# Autodesk Inventor assembly: SE Base Matriz Centelladora DC
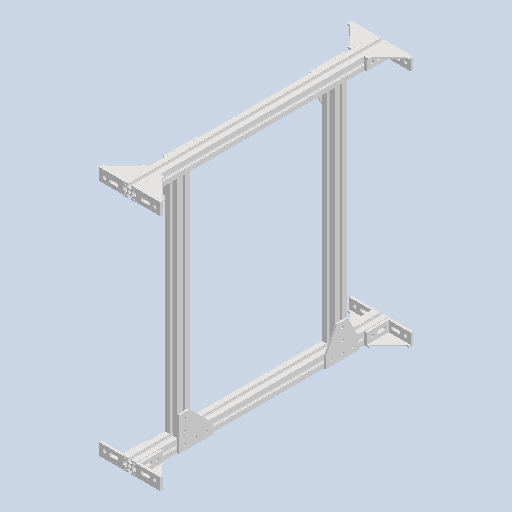
[picture p0: Inventor's stored thumbnail of the model, 512x512]
Saved by Autodesk Inventor 2024.2 (Build 282272000, 272)
## iProperties
Created: 2025-11-13
Part Number: SE Base Matriz Centelladora DC
Document SubType Name: Assembly
Designer: ja.restrepo1
Author: ja.restrepo1
## Documents named in this file (7)
- I:\MICROMECANICA\ALTAS ENERGIAS\Deteccion de Muones\Detectores centelladores\Partes Detector Centellador\SE Base Matriz Centelladora DC\SE Base Matriz Centelladora DC.iam
- I:\MICROMECANICA\ALTAS ENERGIAS\Deteccion de Muones\Detectores centelladores\Partes Detector Centellador\SE Chasis DC\Partes Chasis DC\Perfil 45X45\Perfil 45X45x910.ipt
- I:\MICROMECANICA\ALTAS ENERGIAS\Deteccion de Muones\Detectores centelladores\Partes Detector Centellador\SE Chasis DC\Partes Chasis DC\Perfil 45X45.ipt
- I:\MICROMECANICA\ALTAS ENERGIAS\Deteccion de Muones\Detectores centelladores\Partes Detector Centellador\SE Chasis DC\Partes Chasis DC\Perfil 45X45\Perfil 45X45X810.ipt
- I:\MICROMECANICA\ALTAS ENERGIAS\Deteccion de Muones\Detectores centelladores\Partes Detector Centellador\SE Chasis DC\Partes Chasis DC\Accesorios perfileria\escuadra grande.ipt
- I:\MICROMECANICA\ALTAS ENERGIAS\Deteccion de Muones\Detectores centelladores\Partes Detector Centellador\SE Chasis DC\Partes Chasis DC\Accesorios perfileria\escuadra plana.ipt
- I:\MICROMECANICA\ALTAS ENERGIAS\Deteccion de Muones\Detectores centelladores\Partes Detector Centellador\SE Chasis DC\Partes Chasis DC\Accesorios perfileria\T.ipt
## Components (16 placed, 5 different names)
1. Perfil 45X45x910:1 — Nivelación:19, Nivelación:20, Nivelación:21, Nivelación:22, Nivelación:23, Nivelación:24, Nivelación:25, Nivelación:26
2. Perfil 45X45x910:2 — Nivelación:19, Nivelación:27, Nivelación:28, Nivelación:29, Nivelación:30
3. Perfil 45X45X810:3
4. Perfil 45X45X810:4 — Nivelación:20
5. escuadra grande:1 — Nivelación:23
6. escuadra grande:2 — Nivelación:24
7. escuadra grande:3 — Nivelación:30
8. escuadra grande:4 — Nivelación:26
9. escuadra grande:5 — Nivelación:28
10. escuadra grande:6 — Nivelación:27
11. escuadra grande:7 — Nivelación:25
12. escuadra grande:8 — Nivelación:29
13. escuadra plana:1
14. T:1
15. T:2
16. escuadra plana:2
## Relationships (47: Flush 30, Mate 17)
- [Flush]: Perfil 45X45X810:3 ↔ Perfil 45X45X810:4
- [Flush]: Perfil 45X45X810:3 ↔ Perfil 45X45X810:4
- [Flush]: Perfil 45X45x910:1 ↔ Perfil 45X45X810:4
- [Mate]: Perfil 45X45x910:2 ↔ Perfil 45X45X810:4
- [Flush]: Perfil 45X45x910:2 ↔ Perfil 45X45X810:4
- [Mate]: Perfil 45X45x910:1 ↔ Perfil 45X45X810:3
- [Mate] (-610 mm): Perfil 45X45X810:3 ↔ Perfil 45X45X810:4
- [Flush]: Perfil 45X45x910:1 ↔ escuadra grande:7
- [Mate]: Perfil 45X45x910:1 ↔ escuadra grande:7
- [Mate]: Perfil 45X45x910:1 ↔ escuadra grande:2
- [Mate]: Perfil 45X45x910:1 ↔ escuadra grande:2
- [Flush]: Perfil 45X45x910:1 ↔ escuadra grande:1
- [Mate]: Perfil 45X45x910:1 ↔ escuadra grande:1
- [Flush]: Perfil 45X45x910:1 ↔ escuadra grande:4
- [Mate]: Perfil 45X45x910:1 ↔ escuadra grande:4
- [Flush]: Perfil 45X45x910:2 ↔ escuadra grande:5
- [Mate]: Perfil 45X45x910:2 ↔ escuadra grande:5
- [Flush]: Perfil 45X45x910:2 ↔ escuadra grande:6
- [Mate]: Perfil 45X45x910:2 ↔ escuadra grande:6
- [Flush]: Perfil 45X45x910:2 ↔ escuadra grande:8
- [Mate]: Perfil 45X45x910:2 ↔ escuadra grande:8
- [Flush]: Perfil 45X45x910:2 ↔ escuadra grande:3
- [Mate]: Perfil 45X45x910:2 ↔ escuadra grande:3
- [Mate]: Perfil 45X45X810:4 ↔ escuadra plana:1
- [Flush]: Perfil 45X45x910:1 ↔ escuadra plana:1
- [Flush]: Perfil 45X45X810:4 ↔ escuadra plana:1
- [Mate]: Perfil 45X45X810:3 ↔ T:2
- [Flush]: Perfil 45X45x910:1 ↔ T:2
- [Mate] (-2.5 mm): Perfil 45X45X810:3 ↔ T:2
- [Mate]: Perfil 45X45X810:3 ↔ T:1
- [Flush]: Perfil 45X45x910:2 ↔ T:1
- [Flush]: T:1 ↔ T:2
- [Mate]: Perfil 45X45X810:4 ↔ escuadra plana:2
- [Flush]: Perfil 45X45x910:2 ↔ escuadra plana:2
- [Flush]: Perfil 45X45X810:4 ↔ escuadra plana:2
- Nivelación:19 [Flush]: Perfil 45X45x910:1 ↔ Perfil 45X45x910:2
- Nivelación:20 [Flush] (150 mm): Perfil 45X45x910:1 ↔ Perfil 45X45X810:4
- Nivelación:21 [Flush] (455 mm): Perfil 45X45x910:1
- Nivelación:22 [Flush] (455 mm): Perfil 45X45x910:1
- Nivelación:23 [Flush]: Perfil 45X45x910:1 ↔ escuadra grande:1
- Nivelación:24 [Flush]: Perfil 45X45x910:1 ↔ escuadra grande:2
- Nivelación:25 [Flush]: Perfil 45X45x910:1 ↔ escuadra grande:7
- Nivelación:26 [Flush]: Perfil 45X45x910:1 ↔ escuadra grande:4
- Nivelación:27 [Flush]: Perfil 45X45x910:2 ↔ escuadra grande:6
- Nivelación:28 [Flush]: Perfil 45X45x910:2 ↔ escuadra grande:5
- Nivelación:29 [Flush]: Perfil 45X45x910:2 ↔ escuadra grande:8
- Nivelación:30 [Flush]: Perfil 45X45x910:2 ↔ escuadra grande:3
